# Autodesk Inventor assembly: fullbody
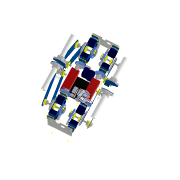
[picture p0: Inventor's stored thumbnail of the model, 180x180]
Saved by Autodesk Inventor 2020.5 (Build 245400000, 400)
## iProperties
Created: 2022-11-17
Part Number: fullbody
Document SubType Name: Assembly
Designer: kanazawakotaro
Author: kanazawakotaro
## Documents named in this file (11)
- C:\Users\Administrator\Documents\kamuy2\kamuy2\fullbody.iam
- C:\Users\Administrator\Documents\kamuy2\kamuy2\VER2.0_MIR_CPY.iam
- C:\Users\Administrator\Documents\kamuy2\kamuy2\VER2.0_MIR_CPY_MIR.iam
- C:\Users\Administrator\Documents\kamuy2\kamuy2\3dprinter\Part1.ipt
- C:\Users\Administrator\Documents\kamuy2\kamuy2\Parts\BGTAB6900VV_Autodesk_Inventor_2020_20221121\AIS2020\BGTAB6900VV.iam
- C:\Users\Administrator\Documents\kamuy2\kamuy2\3dprinter\lipo.ipt
- C:\Users\Administrator\Documents\kamuy2\kamuy2\3dprinter\nuc.ipt
- C:\Users\Administrator\Documents\kamuy2\kamuy2\VER2.0_MIR_CPY_MIR1.iam
- C:\Users\Administrator\Documents\kamuy2\kamuy2\VER2.0_MIR_CPY_MIR_MIR.iam
- C:\Users\Administrator\Documents\kamuy2\kamuy2\3dprinter\Part75.ipt
- C:\Users\Administrator\Desktop\Part76.ipt
## Components (15 placed, 10 different names)
1. VER2.0_MIR_CPY:2 [sub-assembly] — フラッシュ:24, フラッシュ:29, フラッシュ:30, メイト:5, メイト:6
2. VER2.0_MIR_CPY_MIR:2 [sub-assembly] — フラッシュ:20, メイト:4
3. Part1:1 — フラッシュ:20
4. BGTAB6900VV:1 [sub-assembly]
5. BGTAB6900VV:2 [sub-assembly]
6. BGTAB6900VV:3 [sub-assembly]
7. BGTAB6900VV:4 [sub-assembly]
8. lipo:1 — フラッシュ:23, フラッシュ:24, フラッシュ:25, フラッシュ:26, フラッシュ:31, メイト:5
9. lipo:2 — フラッシュ:22, フラッシュ:25
10. nuc:1 — フラッシュ:22, フラッシュ:23, フラッシュ:26
11. VER2.0_MIR_CPY_MIR1:1 [sub-assembly] — メイト:3, フラッシュ:27, フラッシュ:28, フラッシュ:29, フラッシュ:30, フラッシュ:31, フラッシュ:32, メイト:34
12. VER2.0_MIR_CPY_MIR_MIR:1 [sub-assembly] — メイト:3, フラッシュ:27, フラッシュ:28, メイト:4
13. Part75:1 — フラッシュ:32
14. Part76:1 — メイト:34
15. Part76:2 — メイト:6
## Relationships (20: Flush 14, Mate 6)
- [Flush]: VER2.0_MIR_CPY:2 ↔ VER2.0_MIR_CPY_MIR:2
- [Flush]: VER2.0_MIR_CPY:2 ↔ VER2.0_MIR_CPY_MIR:2
- [Mate]: VER2.0_MIR_CPY:2 ↔ VER2.0_MIR_CPY_MIR:2
- フラッシュ:20 [Flush]: VER2.0_MIR_CPY_MIR:2 ↔ Part1:1
- フラッシュ:22 [Flush] (50 mm): lipo:2 ↔ nuc:1
- フラッシュ:23 [Flush] (50 mm): lipo:1 ↔ nuc:1
- フラッシュ:24 [Flush] (30 mm): VER2.0_MIR_CPY:2 ↔ lipo:1
- フラッシュ:25 [Flush]: lipo:1 ↔ lipo:2
- フラッシュ:26 [Flush] (20 mm): lipo:1 ↔ nuc:1
- メイト:3 [Mate]: VER2.0_MIR_CPY_MIR1:1 ↔ VER2.0_MIR_CPY_MIR_MIR:1
- フラッシュ:27 [Flush]: VER2.0_MIR_CPY_MIR1:1 ↔ VER2.0_MIR_CPY_MIR_MIR:1
- フラッシュ:28 [Flush]: VER2.0_MIR_CPY_MIR1:1 ↔ VER2.0_MIR_CPY_MIR_MIR:1
- フラッシュ:29 [Flush]: VER2.0_MIR_CPY:2 ↔ VER2.0_MIR_CPY_MIR1:1
- フラッシュ:30 [Flush]: VER2.0_MIR_CPY:2 ↔ VER2.0_MIR_CPY_MIR1:1
- メイト:4 [Mate] (90 mm): VER2.0_MIR_CPY_MIR:2 ↔ VER2.0_MIR_CPY_MIR_MIR:1
- フラッシュ:31 [Flush]: lipo:1 ↔ VER2.0_MIR_CPY_MIR1:1
- メイト:5 [Mate]: VER2.0_MIR_CPY:2 ↔ lipo:1
- フラッシュ:32 [Flush]: VER2.0_MIR_CPY_MIR1:1 ↔ Part75:1
- メイト:34 [Mate]: VER2.0_MIR_CPY_MIR1:1 ↔ Part76:1
- メイト:6 [Mate]: VER2.0_MIR_CPY:2 ↔ Part76:2
## Named parameters: d20_d16 = 0 mm, d21_d18 = 0 mm, d22_d19 = 0 mm
